# Autodesk Inventor assembly: Assembly1
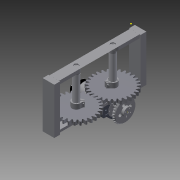
[picture p0: Inventor's stored thumbnail of the model, 180x180]
Saved by Autodesk Inventor 2015 (Build 190159000, 159)
## iProperties
Created: 2014-11-22
Part Number: Assembly1
Document SubType Name: Assembly
Designer: jesse
Author: jesse
## Documents named in this file (14)
- C:\Users\jesse\Desktop\robot\New Pickup\Assembly1.iam
- C:\Users\jesse\Desktop\robot\New Pickup\Top piece.ipt
- C:\Users\jesse\Desktop\robot\New Pickup\Rod.ipt
- C:\Users\jesse\Desktop\robot\New Pickup\roller.ipt
- C:\Users\jesse\Desktop\robot\New Pickup\Assembly1\Design Accelerator\Spur Gears1.iam
- C:\Users\jesse\Desktop\robot\stock parts\tetrix_739376_2pc_motormnt_2013\tetrix_739376_2pc_motormnt_2013-2.iam
- C:\Users\jesse\Desktop\robot\stock parts\am-2964NeveRest\am-2964NeveRest.ipt
- C:\Users\jesse\Desktop\robot\stock parts\tetrix_738007_bevel-1_2013\tetrix_738007_bevel-1_2013.ipt
- C:\Users\jesse\Desktop\robot\stock parts\hub_motor_shaft_2012\hub_motor_shaft_2012.ipt
- C:\Users\jesse\Desktop\robot\stock parts\screw_shcs_6-32_x_0_3125_2012\screw_shcs_6-32_x_0_3125_2012.ipt
- C:\Users\jesse\Desktop\robot\stock parts\tube_clamp_2012\tube_clamp_2012.ipt
- C:\Users\jesse\Desktop\robot\New Pickup\bottom piece.ipt
- C:\Users\jesse\Desktop\robot\New Pickup\side piece.ipt
- C:\Users\jesse\Desktop\robot\stock parts\nylon 1-4-20 nut\nylon 1-4-20 nut.ipt
## Components (30 placed, 13 different names)
1. bottom piece:1 — Mate:1, Mate:2, Flush:1, Flush:2, Flush:6, Mate:63, Mate:64, Mate:65, Mate:66, Mate:67, Mate:68, Mate:69, Mate:71
2. Rod:1 — Mate:2, Flush:2, Mate:11, Mate:13, Mate:17, Mate:70
3. Rod:2 — Mate:1, Flush:1, Mate:10, Mate:14, Mate:72
4. roller:1 — Mate:40, Mate:43, Mate:69, Mate:70
5. roller:2 — Mate:44, Mate:45, Mate:71, Mate:72
6. Spur Gears:1 [sub-assembly] — Mate:10, Mate:11, Mate:16, Mate:18, Mate:46, Mate:47, Mate:48, Mate:49, Mate:50, Mate:51, Mate:52, Mate:53, Mate:54, Mate:55, Mate:56, Mate:58, Mate:59
7. Top piece:3 — Mate:13, Mate:14, Mate:15, Flush:3, Flush:5, Mate:59, Mate:60, Mate:61, Mate:62
8. tetrix_739376_2pc_motormnt_2013-2:1 [sub-assembly] — Mate:15, Flush:3, Mate:20, Flush:4, Flush:5
9. am-2964NeveRest:1 — Mate:19, Mate:20, Flush:4, Mate:21
10. tetrix_738007_bevel-1_2013:1 — Mate:16, Mate:17, Mate:18, Mate:32, Mate:33, Mate:34, Mate:35, Mate:36, Mate:37, Mate:38, Mate:39, Rotation:1, Mate:57
11. tetrix_738007_bevel-1_2013:2 — Mate:19, Mate:22, Mate:23, Mate:24, Mate:25, Mate:26, Mate:27, Mate:28, Mate:29, Mate:30, Mate:31, Rotation:1, Mate:57, Mate:58
12. hub_motor_shaft_2012:1 — Mate:21, Mate:22, Mate:23
13. screw_shcs_6-32_x_0_3125_2012:1 — Mate:24, Mate:31
14. screw_shcs_6-32_x_0_3125_2012:3 — Mate:25, Mate:30
15. screw_shcs_6-32_x_0_3125_2012:4 — Mate:26, Mate:29
16. screw_shcs_6-32_x_0_3125_2012:5 — Mate:27, Mate:28
17. screw_shcs_6-32_x_0_3125_2012:6 — Mate:33, Mate:39
18. screw_shcs_6-32_x_0_3125_2012:7 — Mate:34, Mate:37
19. screw_shcs_6-32_x_0_3125_2012:8 — Mate:35, Mate:36
20. screw_shcs_6-32_x_0_3125_2012:9 — Mate:32, Mate:38
21. tube_clamp_2012:1 — Mate:40, Mate:43, Mate:46
22. tube_clamp_2012:2 — Mate:44, Mate:45, Mate:47, Mate:56
23. screw_shcs_6-32_x_0_3125_2012:10 — Mate:48, Mate:55
24. screw_shcs_6-32_x_0_3125_2012:11 — Mate:51, Mate:53
25. screw_shcs_6-32_x_0_3125_2012:12 — Mate:50, Mate:52
26. screw_shcs_6-32_x_0_3125_2012:13 — Mate:49, Mate:54
27. side piece:1 — Flush:6
28. side piece:2 — Mate:60, Mate:61, Mate:62
29. nylon 1-4-20 nut:1 — Mate:63, Mate:64, Mate:65
30. nylon 1-4-20 nut:2 — Mate:66, Mate:67, Mate:68
## Relationships (69: Mate 62, Flush 6, RelateRotation 1)
- Mate:1: bottom piece:1 ↔ Rod:2
- Mate:2: bottom piece:1 ↔ Rod:1
- Flush:1: bottom piece:1 ↔ Rod:2
- Flush:2: bottom piece:1 ↔ Rod:1
- Mate:10: Rod:2 ↔ Spur Gears:1
- Mate:11: Rod:1 ↔ Spur Gears:1
- Mate:13: Rod:1 ↔ Top piece:3
- Mate:14: Rod:2 ↔ Top piece:3
- Mate:15: Top piece:3 ↔ tetrix_739376_2pc_motormnt_2013-2:1
- Flush:3 (6.35 mm): Top piece:3 ↔ tetrix_739376_2pc_motormnt_2013-2:1
- Mate:16: Spur Gears:1 ↔ tetrix_738007_bevel-1_2013:1
- Mate:17: Rod:1 ↔ tetrix_738007_bevel-1_2013:1
- Mate:18: Spur Gears:1 ↔ tetrix_738007_bevel-1_2013:1
- Mate:19: am-2964NeveRest:1 ↔ tetrix_738007_bevel-1_2013:2
- Mate:20: tetrix_739376_2pc_motormnt_2013-2:1 ↔ am-2964NeveRest:1
- Flush:4: tetrix_739376_2pc_motormnt_2013-2:1 ↔ am-2964NeveRest:1
- Mate:21: am-2964NeveRest:1 ↔ hub_motor_shaft_2012:1
- Mate:22: tetrix_738007_bevel-1_2013:2 ↔ hub_motor_shaft_2012:1
- Mate:23: tetrix_738007_bevel-1_2013:2 ↔ hub_motor_shaft_2012:1
- Mate:24: tetrix_738007_bevel-1_2013:2 ↔ screw_shcs_6-32_x_0_3125_2012:1
- Mate:25: tetrix_738007_bevel-1_2013:2 ↔ screw_shcs_6-32_x_0_3125_2012:3
- Mate:26: tetrix_738007_bevel-1_2013:2 ↔ screw_shcs_6-32_x_0_3125_2012:4
- Mate:27: tetrix_738007_bevel-1_2013:2 ↔ screw_shcs_6-32_x_0_3125_2012:5
- Mate:28: tetrix_738007_bevel-1_2013:2 ↔ screw_shcs_6-32_x_0_3125_2012:5
- Mate:29: tetrix_738007_bevel-1_2013:2 ↔ screw_shcs_6-32_x_0_3125_2012:4
- Mate:30: tetrix_738007_bevel-1_2013:2 ↔ screw_shcs_6-32_x_0_3125_2012:3
- Mate:31: tetrix_738007_bevel-1_2013:2 ↔ screw_shcs_6-32_x_0_3125_2012:1
- Mate:32: tetrix_738007_bevel-1_2013:1 ↔ screw_shcs_6-32_x_0_3125_2012:9
- Mate:33: tetrix_738007_bevel-1_2013:1 ↔ screw_shcs_6-32_x_0_3125_2012:6
- Mate:34: tetrix_738007_bevel-1_2013:1 ↔ screw_shcs_6-32_x_0_3125_2012:7
- Mate:35: tetrix_738007_bevel-1_2013:1 ↔ screw_shcs_6-32_x_0_3125_2012:8
- Mate:36: tetrix_738007_bevel-1_2013:1 ↔ screw_shcs_6-32_x_0_3125_2012:8
- Mate:37: tetrix_738007_bevel-1_2013:1 ↔ screw_shcs_6-32_x_0_3125_2012:7
- Mate:38: tetrix_738007_bevel-1_2013:1 ↔ screw_shcs_6-32_x_0_3125_2012:9
- Mate:39: tetrix_738007_bevel-1_2013:1 ↔ screw_shcs_6-32_x_0_3125_2012:6
- Rotation:1 [RelateRotation] (1 ul): tetrix_738007_bevel-1_2013:1 ↔ tetrix_738007_bevel-1_2013:2
- Flush:5 (38.735 mm): Top piece:3 ↔ tetrix_739376_2pc_motormnt_2013-2:1
- Mate:40: roller:1 ↔ tube_clamp_2012:1
- Mate:43: roller:1 ↔ tube_clamp_2012:1
- Mate:44: roller:2 ↔ tube_clamp_2012:2
- Mate:45: roller:2 ↔ tube_clamp_2012:2
- Mate:46: Spur Gears:1 ↔ tube_clamp_2012:1
- Mate:47: Spur Gears:1 ↔ tube_clamp_2012:2
- Mate:48: Spur Gears:1 ↔ screw_shcs_6-32_x_0_3125_2012:10
- Mate:49: Spur Gears:1 ↔ screw_shcs_6-32_x_0_3125_2012:13
- Mate:50: Spur Gears:1 ↔ screw_shcs_6-32_x_0_3125_2012:12
- Mate:51: Spur Gears:1 ↔ screw_shcs_6-32_x_0_3125_2012:11
- Mate:52: Spur Gears:1 ↔ screw_shcs_6-32_x_0_3125_2012:12
- Mate:53: Spur Gears:1 ↔ screw_shcs_6-32_x_0_3125_2012:11
- Mate:54: Spur Gears:1 ↔ screw_shcs_6-32_x_0_3125_2012:13
- Mate:55: Spur Gears:1 ↔ screw_shcs_6-32_x_0_3125_2012:10
- Mate:56: Spur Gears:1 ↔ tube_clamp_2012:2
- Mate:57 (-33.02 mm): tetrix_738007_bevel-1_2013:1 ↔ tetrix_738007_bevel-1_2013:2
- Mate:58 (33.02 mm): Spur Gears:1 ↔ tetrix_738007_bevel-1_2013:2
- Mate:59 (10.668 mm): Spur Gears:1 ↔ Top piece:3
- Flush:6: bottom piece:1 ↔ side piece:1
- Mate:60: Top piece:3 ↔ side piece:2
- Mate:61: Top piece:3 ↔ side piece:2
- Mate:62: Top piece:3 ↔ side piece:2
- Mate:63: bottom piece:1 ↔ nylon 1-4-20 nut:1
- Mate:64: bottom piece:1 ↔ nylon 1-4-20 nut:1
- Mate:65: bottom piece:1 ↔ nylon 1-4-20 nut:1
- Mate:66: bottom piece:1 ↔ nylon 1-4-20 nut:2
- Mate:67: bottom piece:1 ↔ nylon 1-4-20 nut:2
- Mate:68: bottom piece:1 ↔ nylon 1-4-20 nut:2
- Mate:69: bottom piece:1 ↔ roller:1
- Mate:70: Rod:1 ↔ roller:1
- Mate:71: bottom piece:1 ↔ roller:2
- Mate:72: Rod:2 ↔ roller:2
